# Autodesk Inventor assembly: boe-bot
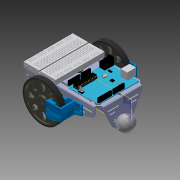
[picture p0: Inventor's stored thumbnail of the model, 180x180]
Saved by Autodesk Inventor 2015 (Build 190159000, 159)
## iProperties
Created: 2015-04-21
Part Number: boe-bot
Document SubType Name: Assembly
Designer: Kyle
Sending System: SolidWorks 2013
Last Author: Branimir
Author: Kyle
## Documents named in this file (15)
- C:\Users\Kyle\Desktop\Programming\cmp-arduino-1678\CAD\sklopovi\Imported Components\boe-bot\boe-bot.iam
- C:\Users\Kyle\Desktop\Programming\cmp-arduino-1678\CAD\sklopovi\Imported Components\boe-bot\boe-bot.ipt
- C:\Users\Kyle\Desktop\Programming\cmp-arduino-1678\CAD\sklopovi\Imported Components\boe-bot\servo motor.ipt
- C:\Users\Kyle\Desktop\Programming\cmp-arduino-1678\CAD\sklopovi\Imported Components\boe-bot\caster.ipt
- C:\Users\Kyle\Desktop\Programming\cmp-arduino-1678\CAD\sklopovi\Imported Components\boe-bot\felga.ipt
- C:\Users\Kyle\Desktop\Programming\cmp-arduino-1678\CAD\sklopovi\Imported Components\boe-bot\guma.ipt
- C:\Users\Kyle\Desktop\Programming\cmp-arduino-1678\CAD\Line Tracker v3.ipt
- C:\Users\Kyle\Desktop\Programming\cmp-arduino-1678\CAD\sklopovi\Imported Components\boe-bot\servo motor_MIR.ipt
- C:\Users\Kyle\Desktop\Programming\cmp-arduino-1678\CAD\sklopovi\Imported Components\boe-bot\felga_MIR1.ipt
- C:\Users\Kyle\Desktop\Programming\cmp-arduino-1678\CAD\sklopovi\Imported Components\boe-bot\guma_MIR1.ipt
- C:\Users\Kyle\Desktop\Programming\cmp-arduino-1678\CAD\Line Tracker v3_MIR.ipt
- C:\Users\Kyle\Desktop\Programming\cmp-arduino-1678\CAD\Imported Components\MiniBreadboard\MiniBreadboard.ipt
- C:\Users\Kyle\Desktop\Programming\cmp-arduino-1678\CAD\Imported Components\Arduino uno\Arduino uno.ipt
- C:\Users\Kyle\Desktop\Programming\cmp-arduino-1678\CAD\Encoder Mount v2.ipt
- C:\Users\Kyle\Desktop\Programming\cmp-arduino-1678\CAD\Encoder Mount v2_MIR.ipt
## Components (14 placed, 14 different names)
1. boe-bot:1 — Mate:2, Flush:4, Mate:4, Flush:7, Flush:8, Mate:5, Flush:9, Mate:6, Mate:7, Mate:9, Mate:10, Mate:11
2. servo motor:1 — Mate:1, Flush:2, Flush:3, Mate:2, Insert:1, Mate:7, Mate:9, Mate:10, Mate:11
3. caster:1
4. felga:3 — Insert:1, Insert:2
5. guma:3 — Insert:2
6. Line Tracker v3:1 — Mate:1, Flush:2, Flush:3
7. servo motor_MIR:1 — Insert:3, Flush:5, Flush:6, Mate:3
8. felga_MIR1:1 — Insert:3, Insert:4
9. guma_MIR1:1 — Insert:4
10. Line Tracker v3_MIR:1 — Flush:5, Flush:6, Mate:3
11. MiniBreadboard:1 — Mate:4, Flush:7, Flush:8
12. Arduino uno:1 — Mate:5, Flush:9
13. Encoder Mount v2:1 — Mate:6
14. Encoder Mount v2_MIR:1
## Relationships (22: Mate 10, Flush 8, Insert 4)
- Mate:1: servo motor:1 ↔ Line Tracker v3:1
- Flush:2: servo motor:1 ↔ Line Tracker v3:1
- Flush:3: servo motor:1 ↔ Line Tracker v3:1
- Mate:2: boe-bot:1 ↔ servo motor:1
- Flush:4 (38.5 mm): boe-bot:1
- Insert:1: servo motor:1 ↔ felga:3
- Insert:2: felga:3 ↔ guma:3
- Insert:3: servo motor_MIR:1 ↔ felga_MIR1:1
- Insert:4: felga_MIR1:1 ↔ guma_MIR1:1
- Flush:5: servo motor_MIR:1 ↔ Line Tracker v3_MIR:1
- Flush:6: servo motor_MIR:1 ↔ Line Tracker v3_MIR:1
- Mate:3: servo motor_MIR:1 ↔ Line Tracker v3_MIR:1
- Mate:4: boe-bot:1 ↔ MiniBreadboard:1
- Flush:7: boe-bot:1 ↔ MiniBreadboard:1
- Flush:8 (2 mm): boe-bot:1 ↔ MiniBreadboard:1
- Mate:5: boe-bot:1 ↔ Arduino uno:1
- Flush:9 (5 mm): boe-bot:1 ↔ Arduino uno:1
- Mate:6: boe-bot:1 ↔ Encoder Mount v2:1
- Mate:7: boe-bot:1 ↔ servo motor:1
- Mate:9 (0.5 mm): boe-bot:1 ↔ servo motor:1
- Mate:10: boe-bot:1 ↔ servo motor:1
- Mate:11 (1 mm): boe-bot:1 ↔ servo motor:1
